# Autodesk Inventor assembly: wheel_shaft_hex_assembly
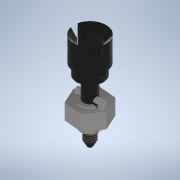
[picture p0: Inventor's stored thumbnail of the model, 180x180]
Saved by Autodesk Inventor 2020 (Build 240168000, 168)
## iProperties
Created: 2019-12-06
Part Number: wheel_shaft_hex_assembly
Document SubType Name: Assembly
Designer: maste
Author: maste
## Documents named in this file (4)
- C:\Users\maste\Documents\GitHub\autobot\robot_model\wheel_shaft_hex_assembly.iam
- C:\Users\maste\Documents\GitHub\autobot\robot_model\RCT-H005.ipt
- C:\Users\maste\Documents\GitHub\autobot\robot_model\RCT-H009_shaft.ipt
- C:\Users\maste\Documents\GitHub\autobot\robot_model\RCT-H009_tuerca.ipt
## Components (3 placed, 3 different names)
1. RCT-H005:1 — Mate:1, Mate:2
2. RCT-H009_shaft:1 — Mate:1
3. RCT-H009_tuerca:1 — Mate:2
## Relationships (2: Mate 2)
- Mate:1: RCT-H005:1 ↔ RCT-H009_shaft:1
- Mate:2: RCT-H005:1 ↔ RCT-H009_tuerca:1
